# Autodesk Inventor assembly: carriage_internal
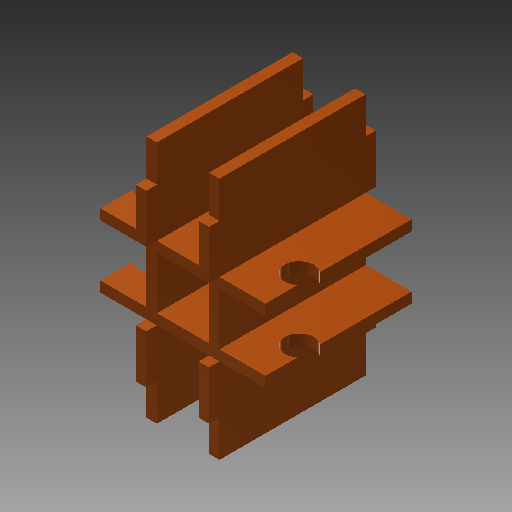
[picture p0: Inventor's stored thumbnail of the model, 512x512]
Saved by Autodesk Inventor 2017 (Build 210142000, 142)
## iProperties
Created: 2015-10-11
Part Number: carriage_internal
Document SubType Name: Assembly
Designer: daniel
Author: daniel
## Documents named in this file (3)
- C:\Users\daniel\Documents\GitHub\cardboard-stage-metric\stage\carriage_internal.iam
- C:\Users\daniel\Documents\GitHub\cardboard-stage-metric\stage\c3.ipt
- C:\Users\daniel\Documents\GitHub\cardboard-stage-metric\stage\c4.ipt
## Components (4 placed, 2 different names)
1. c3:1 — Mate:7, Mate:8, Mate:9
2. c4:1 — Mate:4, Mate:5, Mate:6
3. c3:2 — Mate:1, Mate:2, Mate:3, Mate:4, Mate:5, Mate:6
4. c4:2 — Mate:1, Mate:2, Mate:3, Mate:7, Mate:8, Mate:9
## Relationships (9: Mate 9)
- Mate:1: c3:2 ↔ c4:2
- Mate:2: c3:2 ↔ c4:2
- Mate:3: c3:2 ↔ c4:2
- Mate:4: c4:1 ↔ c3:2
- Mate:5: c4:1 ↔ c3:2
- Mate:6: c4:1 ↔ c3:2
- Mate:7: c3:1 ↔ c4:2
- Mate:8: c3:1 ↔ c4:2
- Mate:9: c3:1 ↔ c4:2
